# Autodesk Inventor assembly: Rear_Train
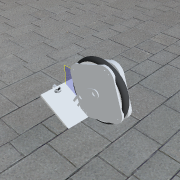
[picture p0: Inventor's stored thumbnail of the model, 180x180]
Saved by Autodesk Inventor 2016 (Build 200138000, 138)
## iProperties
Created: 2015-04-04
Part Number: Rear_Train
Document SubType Name: Assembly
Designer: Yann
Author: Yann
## Documents named in this file (6)
- C:\Users\Yann\Documents\GitHub\BIKAIR_CAD\Source\Rear_Train\Rear_Train.iam
- C:\Users\Yann\Documents\GitHub\BIKAIR_CAD\Source\Rear_Train\Suspension\Rock Shox\Rock Shox.iam
- C:\Users\Yann\Documents\GitHub\BIKAIR_CAD\Source\Rear_Train\Wheel\wheel.iam
- C:\Users\Yann\Documents\GitHub\BIKAIR_CAD\Source\Rear_Train\Swing_Arm.iam
- C:\Users\Yann\Documents\GitHub\BIKAIR_CAD\Source\Rear_Train\Swing_Arm_MIR.iam
- C:\Users\Yann\Documents\GitHub\BIKAIR_CAD\Source\Rear_Train\Suspension\ShockAbsorber.iam
## Components (5 placed, 5 different names)
1. wheel:1 [sub-assembly] — Mate:2, Flush:1
2. Swing_Arm:1 [sub-assembly] — Mate:3, Flush:2
3. Swing_Arm_MIR:1 [sub-assembly] — Flush:3, Mate:4
4. Rock Shox:1 [sub-assembly] — Placage:1
5. ShockAbsorber:1 [sub-assembly] — Mate:5
## Relationships (10: Mate 6, Flush 4)
- Placage:1 [Mate]: Rock Shox:1
- Mate:2: wheel:1
- Flush:1: wheel:1
- Mate:3: Swing_Arm:1
- Flush:2: Swing_Arm:1
- Flush:3: Swing_Arm_MIR:1
- Mate:4: Swing_Arm_MIR:1
- Mate:5: ShockAbsorber:1
- [Flush] (55 mm): Swing_Arm:1 ↔ Swing_Arm_MIR:1
- [Mate]: Swing_Arm:1 ↔ Swing_Arm_MIR:1
## Named parameters: d10_d1 = 0 mm
